# Autodesk Inventor assembly: NP18-12
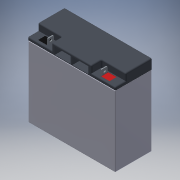
[picture p0: Inventor's stored thumbnail of the model, 180x180]
Saved by Autodesk Inventor 2016 SP1 (Build 200210100, 210)
## iProperties
Category: Electrical
Company: Autodesk Inc.
Created: 2014-12-10
Part Number: NP18-12
Document SubType Name: Assembly
Designer: Autodesk
Description: Battery, ,12 volt, 18 AH, Non-spillable
Mass: 8469.99 g
Surface Area: 1482.32 cm^2
Volume: 2177.92 cm^3
Density: 3.88903 g/cm^3
Author: Autodesk Inc.
## Documents named in this file (3)
- C:\snobotics\autodesk\2015\FRC_KOP_2015\Electrical\ELEC_Battery_NP18-12B.iam
- C:\snobotics\autodesk\2015\FRC_KOP_2015\Electrical\Parts\Electrical_Yuasa_NP18-12_Top.ipt
- C:\snobotics\autodesk\2015\FRC_KOP_2015\Electrical\Parts\Electrical_Yuasa_Np18-12_Middle.ipt
## Components (2 placed, 2 different names)
1. Electrical_Yuasa_NP18-12_Top:1 — Flush:1
2. Electrical_Yuasa_Np18-12_Middle:1 — Flush:1
## Relationships (1: Flush 1)
- Flush:1: Electrical_Yuasa_NP18-12_Top:1 ↔ Electrical_Yuasa_Np18-12_Middle:1
